# Autodesk Inventor assembly: sla2216
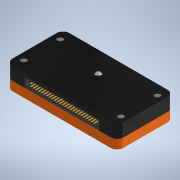
[picture p0: Inventor's stored thumbnail of the model, 180x180]
Saved by Autodesk Inventor 2021 (Build 250183000, 183)
## iProperties
Created: 2022-04-04
Part Number: sla2216
Document SubType Name: Assembly
Designer: Staňa
Author: Staňa
## Documents named in this file (6)
- D:\Projects\Hardware\sla2216\mech\sla2216.iam
- D:\Projects\Hardware\sla2216\mech\sla2216_pcb.iam
- D:\Projects\Hardware\sla2216\mech\casing-bot.ipt
- D:\Projects\Hardware\sla2216\mech\casing-top.ipt
- D:\Projects\Hardware\sla2216\mech\970080365 (rev1).ipt
- D:\Projects\Hardware\sla2216\mech\97790603111 (rev1).ipt
## Components (11 placed, 5 different names)
1. sla2216_pcb:1 [sub-assembly] — Mate:1, Flush:1, Flush:2, Flush:3, Mate:2, Mate:3, Mate:4, Mate:5
2. casing-bot:1 — Flush:4
3. casing-top:1 — Flush:4, Mate:6, Mate:7, Mate:8, Mate:9
4. 970080365 (rev1):1 — Mate:2
5. 970080365 (rev1):2 — Mate:4
6. 970080365 (rev1):3 — Mate:3
7. 970080365 (rev1):4 — Mate:5
8. 97790603111 (rev1):1 — Mate:6
9. 97790603111 (rev1):2 — Mate:7
10. 97790603111 (rev1):3 — Mate:9
11. 97790603111 (rev1):4 — Mate:8
## Relationships (13: Mate 9, Flush 4)
- Mate:1: sla2216_pcb:1
- Flush:1: sla2216_pcb:1
- Flush:2: sla2216_pcb:1
- Flush:3: sla2216_pcb:1
- Flush:4: casing-bot:1 ↔ casing-top:1
- Mate:2: sla2216_pcb:1 ↔ 970080365 (rev1):1
- Mate:3: sla2216_pcb:1 ↔ 970080365 (rev1):3
- Mate:4: sla2216_pcb:1 ↔ 970080365 (rev1):2
- Mate:5: sla2216_pcb:1 ↔ 970080365 (rev1):4
- Mate:6: casing-top:1 ↔ 97790603111 (rev1):1
- Mate:7: casing-top:1 ↔ 97790603111 (rev1):2
- Mate:8: casing-top:1 ↔ 97790603111 (rev1):4
- Mate:9: casing-top:1 ↔ 97790603111 (rev1):3
